# Autodesk Inventor assembly: A001
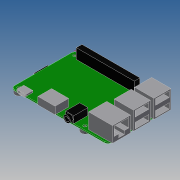
[picture p0: Inventor's stored thumbnail of the model, 180x180]
Saved by Autodesk Inventor 2017 (Build 210142000, 142)
## iProperties
Created: 2018-10-05
Part Number: A001
Document SubType Name: Assembly
Designer: Gilles Mottiez
Description: Raspberry pi 3B
Author: Gilles Mottiez
## Documents named in this file (14)
- C:\Users\Gilles Mottiez\Documents\HES\I5_6\PGA\inventor\rpi3b.iam
- rpi3b.iam
- C:\Users\Gilles Mottiez\Documents\HES\I5_6\PGA\inventor\rpi.ipt
- C:\Users\Gilles Mottiez\Documents\HES\I5_6\PGA\inventor\2usb.ipt
- C:\Users\Gilles Mottiez\Documents\HES\I5_6\PGA\inventor\ethernet.ipt
- C:\Users\Gilles Mottiez\Documents\HES\I5_6\PGA\inventor\spacer_rpi.ipt
- C:\Users\Gilles Mottiez\Documents\HES\I5_6\PGA\inventor\sd.ipt
- C:\Users\Gilles Mottiez\Documents\HES\I5_6\PGA\inventor\hdmi.ipt
- C:\Users\Gilles Mottiez\Documents\HES\I5_6\PGA\inventor\gpio_rpi.ipt
- gpio_rpi.ipt
- C:\Users\Gilles Mottiez\Documents\HES\I5_6\PGA\inventor\micro_usb_connecteur.ipt
- micro_usb_connecteur.ipt
- C:\Users\Gilles Mottiez\Documents\HES\I5_6\PGA\inventor\port_jack_rpi.ipt
- port_jack_rpi.ipt
## Components (13 placed, 9 different names)
1. rpi:1 — Placage:1, Affleurement:1, Placage:2, Affleurement:3, Placage:4, Affleurement:5, Logement:1, Logement:2, Logement:3, Logement:4, Placage:5, Affleurement:6, Affleurement:7, Placage:6, Affleurement:8, Affleurement:9, Placage:7, Affleurement:10, Affleurement:11, Placage:8, Affleurement:12, Affleurement:13, Placage:9, Affleurement:14, Affleurement:15
2. 2usb:1 — Placage:1, Affleurement:1, Affleurement:2, Affleurement:3, Placage:3
3. 2usb:2 — Placage:2, Affleurement:2, Placage:3, Affleurement:4
4. ethernet:1 — Placage:4, Affleurement:4, Affleurement:5
5. spacer_rpi:1 — Logement:2
6. spacer_rpi:2 — Logement:1
7. spacer_rpi:3 — Logement:3
8. spacer_rpi:4 — Logement:4
9. sd:1 — Placage:5, Affleurement:6, Affleurement:7
10. hdmi:1 — Placage:6, Affleurement:8, Affleurement:9
11. gpio_rpi:1 — Placage:7, Affleurement:10, Affleurement:11
12. micro_usb_connecteur:1 — Placage:8, Affleurement:12, Affleurement:13
13. port_jack_rpi:1 — Placage:9, Affleurement:14, Affleurement:15
## Relationships (28: Flush 15, Mate 9, Insert 4)
- Placage:1 [Mate]: rpi:1 ↔ 2usb:1
- Affleurement:1 [Flush] (-2 mm): rpi:1 ↔ 2usb:1
- Placage:2 [Mate]: rpi:1 ↔ 2usb:2
- Affleurement:2 [Flush]: 2usb:1 ↔ 2usb:2
- Affleurement:3 [Flush] (2.5 mm): rpi:1 ↔ 2usb:1
- Placage:3 [Mate] (3 mm): 2usb:1 ↔ 2usb:2
- Placage:4 [Mate]: rpi:1 ↔ ethernet:1
- Affleurement:4 [Flush]: 2usb:2 ↔ ethernet:1
- Affleurement:5 [Flush] (2 mm): rpi:1 ↔ ethernet:1
- Logement:1 [Insert]: rpi:1 ↔ spacer_rpi:2
- Logement:2 [Insert]: rpi:1 ↔ spacer_rpi:1
- Logement:3 [Insert]: rpi:1 ↔ spacer_rpi:3
- Logement:4 [Insert]: rpi:1 ↔ spacer_rpi:4
- Placage:5 [Mate]: rpi:1 ↔ sd:1
- Affleurement:6 [Flush] (22 mm): rpi:1 ↔ sd:1
- Affleurement:7 [Flush] (-2 mm): rpi:1 ↔ sd:1
- Placage:6 [Mate]: rpi:1 ↔ hdmi:1
- Affleurement:8 [Flush] (-1.5 mm): rpi:1 ↔ hdmi:1
- Affleurement:9 [Flush] (25 mm): rpi:1 ↔ hdmi:1
- Placage:7 [Mate]: rpi:1 ↔ gpio_rpi:1
- Affleurement:10 [Flush] (1 mm): rpi:1 ↔ gpio_rpi:1
- Affleurement:11 [Flush] (7.2 mm): rpi:1 ↔ gpio_rpi:1
- Placage:8 [Mate]: rpi:1 ↔ micro_usb_connecteur:1
- Affleurement:12 [Flush] (6.75 mm): rpi:1 ↔ micro_usb_connecteur:1
- Affleurement:13 [Flush] (-1.7 mm): rpi:1 ↔ micro_usb_connecteur:1
- Placage:9 [Mate]: rpi:1 ↔ port_jack_rpi:1
- Affleurement:14 [Flush]: rpi:1 ↔ port_jack_rpi:1
- Affleurement:15 [Flush] (30 mm): rpi:1 ↔ port_jack_rpi:1
